# Autodesk Inventor assembly: 1_Body_Cam1
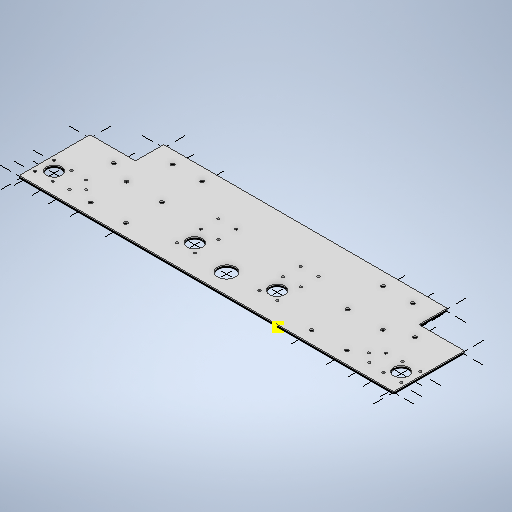
[picture p0: Inventor's stored thumbnail of the model, 512x512]
Saved by Autodesk Inventor 2026.1 (Build 301233000, 233)
## iProperties
Created: 2025-08-16
Part Number: 1_Body_Cam1
Document SubType Name: Assembly
Designer: chris
Author: chris
## Documents named in this file (2)
- C:\Users\chris\Documents\Inventor\RHp_Humanoid_ver1\Cam\Body\1.5T\Assembly\1_Body_Cam1.iam
- C:\Users\chris\Documents\Inventor\RHp_Humanoid_ver1\Cam\Body\1.5T\Part\body_main_frame.ipt
## Components (1 placed, 1 different names)
1. body_main_frame:1 — Mate:1, Mate:2, Flush:1
## Relationships (3: Mate 2, Flush 1)
- Mate:1: body_main_frame:1
- Mate:2: body_main_frame:1
- Flush:1: body_main_frame:1
